# Autodesk Inventor assembly: robot
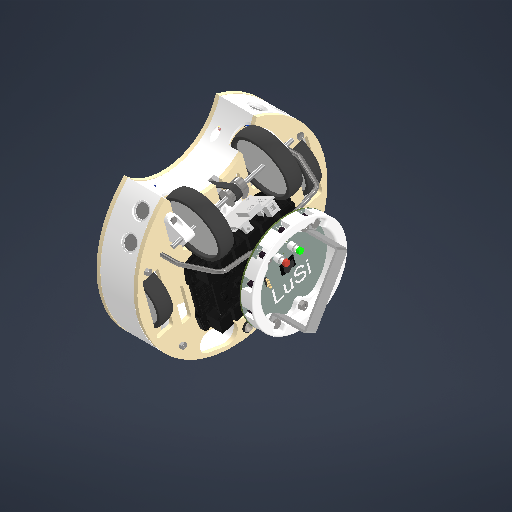
[picture p0: Inventor's stored thumbnail of the model, 512x512]
Saved by Autodesk Inventor 2026.1 (Build 301233000, 233)
## iProperties
Created: 2026-04-20
Part Number: robot
Document SubType Name: Assembly
Designer: Familie
Author: Familie
## Documents named in this file (42)
- C:\Users\Familie\Documents\Luka\Robocup Soccer\Wien\final\robot.iam
- C:\Users\Familie\Documents\Luka\Robocup Soccer\Inventor nach Nürnberg\ball caster.ipt
- C:\Users\Familie\Documents\Luka\Robocup Soccer\Inventor nach Nürnberg\Auriga Steuerboard.ipt
- C:\Users\Familie\Documents\Luka\Robocup Soccer\Inventor nach Nürnberg\Antriebs Rad.ipt
- C:\Users\Familie\Documents\Luka\Robocup Soccer\Inventor nach Nürnberg\Fahrmotor.ipt
- C:\Users\Familie\Documents\Luka\Robocup Soccer\Inventor nach Nürnberg\Mittlere Platte.ipt
- C:\Users\Familie\Documents\Luka\Robocup Soccer\Inventor nach Nürnberg\Grundplatte.ipt
- C:\Users\Familie\Documents\Luka\Robocup Soccer\Inventor nach Nürnberg\Griffroboter.ipt
- C:\Users\Familie\Documents\Luka\Robocup Soccer\Inventor nach Nürnberg\Ultraschalsensor.ipt
- C:\Users\Familie\Documents\Luka\Robocup Soccer\Inventor nach Nürnberg\Umrandung.ipt
- C:\Users\Familie\Documents\Luka\Robocup Soccer\Inventor nach Nürnberg\Halter Ball Caster.ipt
- C:\Users\Familie\Documents\Luka\Robocup Soccer\Inventor nach Nürnberg\IR-Platte.iam
- C:\Users\Familie\Documents\Luka\Robocup Soccer\Inventor nach Nürnberg\Motor Halter.ipt
- C:\Users\Familie\Documents\Inventor\Content Center Files\R2026\de-DE\AS 1110\AS 1110 - M3 x 8.ipt
- C:\Users\Familie\Documents\Inventor\Content Center Files\R2026\de-DE\ANSI B18.2.4.2M\ANSI B18.2.4.2M - M3x0,5 - 5,5.ipt
- C:\Users\Familie\Documents\Inventor\Content Center Files\R2026\de-DE\AS 1110\AS 1110 - M3 x 10.ipt
- C:\Users\Familie\Documents\Inventor\Content Center Files\R2026\de-DE\AS 1110\AS 1110 - M4 x 12.ipt
- C:\Users\Familie\Documents\Inventor\Content Center Files\R2026\de-DE\ANSI B18.2.4.2M\ANSI B18.2.4.2M - M4x0,7 - 7.ipt
- C:\Users\Familie\Documents\Inventor\Content Center Files\R2026\de-DE\AS 1427(03)\AS 1427 - M3 x 6(1).ipt
- C:\Users\Familie\Documents\Luka\KiCad\IR-Platte\Roboter neu\Roboter neu\blue led.ipt
- C:\Users\Familie\Documents\Luka\Robocup Soccer\Inventor nach Nürnberg\LDR\LDR\LDR.ipt
- C:\Users\Familie\Documents\Luka\Robocup Soccer\Inventor nach Nürnberg\Dribbler Motor Halter Oberteil.ipt
- C:\Users\Familie\Documents\Luka\Robocup Soccer\Inventor nach Nürnberg\Dribbler Motor Halter Unterteil.ipt
- C:\Users\Familie\Documents\Luka\Robocup Soccer\Inventor nach Nürnberg\Dribbler Motor.ipt
- C:\Users\Familie\Documents\Luka\Robocup Soccer\Inventor nach Nürnberg\Zahnriemen Rad.ipt
- C:\Users\Familie\Documents\Luka\Robocup Soccer\Inventor\Zahnriemen.ipt
- C:\Users\Familie\Documents\Luka\Robocup Soccer\Inventor nach Nürnberg\Stange Dribbler.ipt
- C:\Users\Familie\Documents\Luka\Robocup Soccer\Inventor nach Nürnberg\Stange Hinten.ipt
- C:\Users\Familie\Documents\Luka\Robocup Soccer\Inventor nach Nürnberg\Stange Vorne.ipt
- C:\Users\Familie\Documents\Luka\Robocup Soccer\Inventor nach Nürnberg\Halter Rolle.ipt
- C:\Users\Familie\Documents\Inventor\Content Center Files\R2026\de-DE\AS 1427(03)\AS 1427 - M3 x 5(1).ipt
- C:\Users\Familie\Documents\Luka\Robocup Soccer\Inventor nach Nürnberg\IR-Blocker.ipt
- C:\Users\Familie\Documents\Inventor\Content Center Files\R2026\de-DE\AS 1110\AS 1110 - M3 x 6.ipt
- C:\Users\Familie\Documents\Luka\Robocup Soccer\Inventor nach Nürnberg\Buchse\Buchse\Buchse.ipt
- C:\Users\Familie\Documents\Luka\Robocup Soccer\Inventor nach Nürnberg\Taster grün.ipt
- C:\Users\Familie\Documents\Luka\Robocup Soccer\Inventor nach Nürnberg\Taster rot.ipt
- C:\Users\Familie\Documents\Luka\Robocup Soccer\Inventor nach Nürnberg\Kippschalter\Kippschalter\Kippschalter.ipt
- C:\Users\Familie\Documents\Inventor\Content Center Files\R2026\de-DE\AS 1110\AS 1110 - M3 x 12.ipt
- C:\Users\Familie\Documents\Inventor\Content Center Files\R2026\de-DE\ANSI B18.2.4.2M\ANSI B18.2.4.2M - M3,5x0,6 - 6.ipt
- C:\Users\Familie\Documents\Luka\Robocup Soccer\Inventor nach Nürnberg\Halter Pixy.ipt
- C:\Users\Familie\Documents\Luka\Robocup Soccer\Inventor nach Nürnberg\Pixy2.ipt
- C:\Users\Familie\Documents\Luka\Robocup Soccer\Inventor nach Nürnberg\Obere Platte.ipt
## Components (107 placed, 41 different names)
1. ball caster:1 — Einfügen:22, Tangential:1, Einfügen:23, Einfügen:24
2. Auriga Steuerboard:1 — Einfügen:69, Winkel:11
3. Antriebs Rad:1 — Einfügen:52
4. Antriebs Rad:2 — Einfügen:51
5. Fahrmotor:1 — Einfügen:45, Einfügen:46, Einfügen:51
6. Fahrmotor:2 — Einfügen:43, Einfügen:44, Einfügen:52
7. Mittlere Platte:1 — Einfügen:62, Einfügen:63, Einfügen:64, Einfügen:65, Einfügen:66, Einfügen:67, Einfügen:68, Einfügen:69, Einfügen:70, Einfügen:72, Winkel:11, Einfügen:74, Einfügen:75, Einfügen:80, Einfügen:81, Einfügen:82, Einfügen:83, Einfügen:89, Einfügen:91, Winkel:12, Einfügen:93, Einfügen:96, Einfügen:101, Einfügen:102, Einfügen:103, Einfügen:104, Einfügen:113, Einfügen:115, Einfügen:117, Einfügen:119, Einfügen:120, Einfügen:121
8. Grundplatte:1 — Passend:1, Passend:2, Passend:3, Passend:4, Passend:5, Passend:6, Passend:7, Passend:8, Passend:9, Passend:10, Passend:11, Passend:12, Einfügen:20, Einfügen:21, Einfügen:25, Einfügen:26, Einfügen:31, Einfügen:32, Einfügen:33, Einfügen:34, Einfügen:35, Einfügen:36, Einfügen:37, Einfügen:38
9. Griffroboter:1 — Einfügen:107, Tangential:8, Einfügen:108, Einfügen:109
10. Umrandung:1 — Passend:1, Passend:12, Passend:13, Passend:14, Winkel:1, Winkel:2, Winkel:3, Winkel:4, Winkel:5, Einfügen:53, Passend:15, Einfügen:54, Passend:16, Einfügen:55, Einfügen:56, Einfügen:57, Einfügen:58, Einfügen:59, Einfügen:60, Einfügen:61, Winkel:6, Winkel:7, Winkel:8, Winkel:9, Winkel:10, Einfügen:62, Einfügen:63
11. Halter Ball Caster:1 — Einfügen:20, Einfügen:21, Einfügen:22, Tangential:1
12. IR-Platte:1 [sub-assembly] — Einfügen:91, Winkel:12, Tangential:5, Tangential:6, Passend:18, Tangential:7, Einfügen:105, Einfügen:106, Passend:20, Passend:21, Passend:22, Einfügen:122
13. Motor Halter:1 — Einfügen:33, Einfügen:34, Einfügen:43, Einfügen:44, Einfügen:49, Einfügen:50
14. Motor Halter:2 — Einfügen:31, Einfügen:32, Einfügen:45, Einfügen:46, Einfügen:47, Einfügen:48
15. AS 1110 - Metrisch M3 x 8:1 — Einfügen:60, Winkel:6
16. AS 1110 - Metrisch M3 x 8:2 — Einfügen:59, Winkel:10
17. AS 1110 - Metrisch M3 x 8:3 — Einfügen:57, Winkel:9
18. AS 1110 - Metrisch M3 x 8:4 — Einfügen:58, Winkel:8
19. AS 1110 - Metrisch M3 x 8:5 — Passend:4, Passend:8, Passend:14, Einfügen:3
20. AS 1110 - Metrisch M3 x 8:6 — Passend:3, Passend:9, Einfügen:18
21. AS 1110 - Metrisch M3 x 8:7 — Passend:2, Passend:10, Passend:13, Einfügen:17
22. AS 1110 - Metrisch M3 x 8:8 — Einfügen:61, Winkel:7
23. AS 1110 - Metrisch M3 x 8:9 — Passend:6, Passend:7, Einfügen:2
24. AS 1110 - Metrisch M3 x 8:10 — Passend:5, Passend:11, Einfügen:19
25. ANSI B18.2.4.2M M3x0,5:1 — Einfügen:68
26. ANSI B18.2.4.2M M3x0,5:2 — Einfügen:66
27. ANSI B18.2.4.2M M3x0,5:3 — Einfügen:67
28. ANSI B18.2.4.2M M3x0,5:4 — Einfügen:65
29. ANSI B18.2.4.2M M3x0,5:5 — Einfügen:64
30. ANSI B18.2.4.2M M3x0,5:6 — Einfügen:19, Winkel:1
31. ANSI B18.2.4.2M M3x0,5:7 — Einfügen:2, Winkel:5
32. ANSI B18.2.4.2M M3x0,5:8 — Einfügen:17, Winkel:2
33. ANSI B18.2.4.2M M3x0,5:9 — Einfügen:3, Winkel:4
34. ANSI B18.2.4.2M M3x0,5:10 — Einfügen:18, Winkel:3
35. ANSI B18.2.4.2M M3x0,5:11 — Einfügen:28
36. ANSI B18.2.4.2M M3x0,5:12 — Einfügen:30
37. ANSI B18.2.4.2M M3x0,5:13 — Einfügen:29
38. ANSI B18.2.4.2M M3x0,5:14 — Einfügen:27
39. AS 1110 - Metrisch M3 x 10:1 — Einfügen:25, Einfügen:27
40. AS 1110 - Metrisch M3 x 10:2 — Einfügen:26, Einfügen:28
41. AS 1110 - Metrisch M3 x 8:11 — Einfügen:24, Einfügen:29
42. AS 1110 - Metrisch M3 x 8:12 — Einfügen:23, Einfügen:30
43. AS 1110 - Metrisch M4 x 12:1 — Einfügen:35, Einfügen:39
44. AS 1110 - Metrisch M4 x 12:2 — Einfügen:36, Einfügen:40
45. AS 1110 - Metrisch M4 x 12:3 — Einfügen:37, Einfügen:41
46. AS 1110 - Metrisch M4 x 12:4 — Einfügen:38, Einfügen:42
47. ANSI B18.2.4.2M M4x0,7:1 — Einfügen:39
48. ANSI B18.2.4.2M M4x0,7:2 — Einfügen:40
49. ANSI B18.2.4.2M M4x0,7:3 — Einfügen:41
50. ANSI B18.2.4.2M M4x0,7:4 — Einfügen:42
51. AS 1427 - Metrisch M3 x 6:1 — Einfügen:48
52. AS 1427 - Metrisch M3 x 6:2 — Einfügen:47
53. AS 1427 - Metrisch M3 x 6:3 — Einfügen:49
54. AS 1427 - Metrisch M3 x 6:4 — Einfügen:50
55. Ultraschalsensor:3 — Einfügen:54, Passend:16
56. Ultraschalsensor:4 — Einfügen:53, Passend:15
57. blue led:1 — Einfügen:55
58. LDR:1 — Einfügen:56
59. AS 1110 - Metrisch M3 x 10:3 — Einfügen:70, Einfügen:71
60. AS 1110 - Metrisch M3 x 10:4 — Einfügen:72, Einfügen:73
61. ANSI B18.2.4.2M M3x0,5:15 — Einfügen:71
62. ANSI B18.2.4.2M M3x0,5:16 — Einfügen:73
63. Dribbler Motor Halter Oberteil:1 — Einfügen:74, Einfügen:75, Passend:17, Fluchtend:1, Fluchtend:2
64. Dribbler Motor Halter Unterteil:1 — Passend:17, Fluchtend:1, Fluchtend:2, Einfügen:76, Tangential:2, Einfügen:78, Einfügen:79
65. Dribbler Motor:1 — Einfügen:76, Tangential:2, Einfügen:77
66. Zahnriemen Rad:1 — Einfügen:87, Einfügen:88
67. Zahnriemen Rad:2 — Einfügen:77, Tangential:3
68. Zahnriemen:1 — Einfügen:88, Tangential:3
69. Stange Dribbler:1 — Einfügen:84, Einfügen:85, Einfügen:86, Einfügen:87
70. Stange Hinten:1 — Einfügen:96, Tangential:7, Einfügen:97, Einfügen:98
71. Stange Vorne:1 — Einfügen:89, Tangential:5, Passend:19, Einfügen:95, Einfügen:99
72. Halter Rolle:1 — Einfügen:80, Einfügen:81, Einfügen:84, Einfügen:112, Einfügen:114
73. Halter Rolle:2 — Einfügen:82, Einfügen:83, Einfügen:116, Einfügen:118
74. Antriebs Rad:3 — Einfügen:85
75. Antriebs Rad:4 — Einfügen:86
76. AS 1427 - Metrisch M3 x 5:1 — Einfügen:78
77. AS 1427 - Metrisch M3 x 5:2 — Einfügen:79
78. Stange Vorne:2 — Einfügen:93, Tangential:6, Einfügen:94, Einfügen:100
79. ANSI B18.2.4.2M M4x0,7:5 — Einfügen:94
80. ANSI B18.2.4.2M M4x0,7:6 — Einfügen:95
81. ANSI B18.2.4.2M M4x0,7:7 — Einfügen:99
82. ANSI B18.2.4.2M M4x0,7:8 — Einfügen:98
83. ANSI B18.2.4.2M M4x0,7:9 — Einfügen:97
84. ANSI B18.2.4.2M M4x0,7:10 — Einfügen:100
85. IR-Blocker:1 — Passend:18, Passend:19, Einfügen:107, Tangential:8
86. AS 1110 - Metrisch M3 x 6:1 — Einfügen:102
87. AS 1110 - Metrisch M3 x 6:2 — Einfügen:101
88. Buchse:1 — Einfügen:104
89. Buchse:2 — Einfügen:103
90. Taster grün:1 — Einfügen:105
91. Taster rot:1 — Einfügen:106
92. Kippschalter:1 — Passend:20, Passend:21, Passend:22, Winkel:13
93. ANSI B18.2.4.2M M4x0,7:11 — Einfügen:110
94. ANSI B18.2.4.2M M4x0,7:12 — Einfügen:111
95. AS 1110 - Metrisch M4 x 12:5 — Einfügen:108, Einfügen:110
96. AS 1110 - Metrisch M4 x 12:6 — Einfügen:109, Einfügen:111
97. AS 1110 - Metrisch M3 x 12:1 — Einfügen:112
98. AS 1110 - Metrisch M3 x 12:2 — Einfügen:114
99. AS 1110 - Metrisch M3 x 12:3 — Einfügen:116
100. AS 1110 - Metrisch M3 x 12:4 — Einfügen:118
101. ANSI B18.2.4.2M M3,5x0,6:1 — Einfügen:113
102. ANSI B18.2.4.2M M3,5x0,6:2 — Einfügen:117
103. ANSI B18.2.4.2M M3,5x0,6:3 — Einfügen:115
104. ANSI B18.2.4.2M M3,5x0,6:4 — Einfügen:119
105. Halter Pixy:1 — Einfügen:120, Einfügen:121, Passend:23, Passend:24
106. Pixy2:1 — Passend:23, Passend:24
107. Obere Platte:1 — Einfügen:122, Winkel:13
## Relationships (152: Insert 106, Mate 24, Angle 13, Tangent 7, Flush 2)
- Passend:1 [Mate]: Grundplatte:1 ↔ Umrandung:1
- Passend:2 [Mate]: Grundplatte:1 ↔ AS 1110 - Metrisch M3 x 8:7
- Passend:3 [Mate]: Grundplatte:1 ↔ AS 1110 - Metrisch M3 x 8:6
- Passend:4 [Mate]: Grundplatte:1 ↔ AS 1110 - Metrisch M3 x 8:5
- Passend:5 [Mate]: Grundplatte:1 ↔ AS 1110 - Metrisch M3 x 8:10
- Passend:6 [Mate]: Grundplatte:1 ↔ AS 1110 - Metrisch M3 x 8:9
- Passend:7 [Mate]: Grundplatte:1 ↔ AS 1110 - Metrisch M3 x 8:9
- Passend:8 [Mate]: Grundplatte:1 ↔ AS 1110 - Metrisch M3 x 8:5
- Passend:9 [Mate]: Grundplatte:1 ↔ AS 1110 - Metrisch M3 x 8:6
- Passend:10 [Mate]: Grundplatte:1 ↔ AS 1110 - Metrisch M3 x 8:7
- Passend:11 [Mate]: Grundplatte:1 ↔ AS 1110 - Metrisch M3 x 8:10
- Passend:12 [Mate]: Grundplatte:1 ↔ Umrandung:1
- Passend:13 [Mate]: Umrandung:1 ↔ AS 1110 - Metrisch M3 x 8:7
- Passend:14 [Mate]: Umrandung:1 ↔ AS 1110 - Metrisch M3 x 8:5
- Einfügen:2 [Insert]: AS 1110 - Metrisch M3 x 8:9 ↔ ANSI B18.2.4.2M M3x0,5:7
- Einfügen:17 [Insert]: AS 1110 - Metrisch M3 x 8:7 ↔ ANSI B18.2.4.2M M3x0,5:8
- Einfügen:3 [Insert]: AS 1110 - Metrisch M3 x 8:5 ↔ ANSI B18.2.4.2M M3x0,5:9
- Einfügen:18 [Insert]: AS 1110 - Metrisch M3 x 8:6 ↔ ANSI B18.2.4.2M M3x0,5:10
- Einfügen:19 [Insert]: AS 1110 - Metrisch M3 x 8:10 ↔ ANSI B18.2.4.2M M3x0,5:6
- Winkel:1 [Angle] (0 deg): Umrandung:1 ↔ ANSI B18.2.4.2M M3x0,5:6
- Winkel:2 [Angle] (0 deg): Umrandung:1 ↔ ANSI B18.2.4.2M M3x0,5:8
- Winkel:3 [Angle] (0 deg): Umrandung:1 ↔ ANSI B18.2.4.2M M3x0,5:10
- Winkel:4 [Angle] (0 deg): Umrandung:1 ↔ ANSI B18.2.4.2M M3x0,5:9
- Winkel:5 [Angle] (0 deg): Umrandung:1 ↔ ANSI B18.2.4.2M M3x0,5:7
- Einfügen:20 [Insert]: Grundplatte:1 ↔ Halter Ball Caster:1
- Einfügen:21 [Insert]: Grundplatte:1 ↔ Halter Ball Caster:1
- Einfügen:22 [Insert]: ball caster:1 ↔ Halter Ball Caster:1
- Tangential:1 (-3 mm): ball caster:1 ↔ Halter Ball Caster:1
- Einfügen:23 [Insert]: ball caster:1 ↔ AS 1110 - Metrisch M3 x 8:12
- Einfügen:24 [Insert]: ball caster:1 ↔ AS 1110 - Metrisch M3 x 8:11
- Einfügen:25 [Insert]: Grundplatte:1 ↔ AS 1110 - Metrisch M3 x 10:1
- Einfügen:26 [Insert]: Grundplatte:1 ↔ AS 1110 - Metrisch M3 x 10:2
- Einfügen:27 [Insert]: ANSI B18.2.4.2M M3x0,5:14 ↔ AS 1110 - Metrisch M3 x 10:1
- Einfügen:28 [Insert]: ANSI B18.2.4.2M M3x0,5:11 ↔ AS 1110 - Metrisch M3 x 10:2
- Einfügen:29 [Insert]: ANSI B18.2.4.2M M3x0,5:13 ↔ AS 1110 - Metrisch M3 x 8:11
- Einfügen:30 [Insert]: ANSI B18.2.4.2M M3x0,5:12 ↔ AS 1110 - Metrisch M3 x 8:12
- Einfügen:31 [Insert]: Grundplatte:1 ↔ Motor Halter:2
- Einfügen:32 [Insert]: Grundplatte:1 ↔ Motor Halter:2
- Einfügen:33 [Insert]: Grundplatte:1 ↔ Motor Halter:1
- Einfügen:34 [Insert]: Grundplatte:1 ↔ Motor Halter:1
- Einfügen:35 [Insert]: Grundplatte:1 ↔ AS 1110 - Metrisch M4 x 12:1
- Einfügen:36 [Insert]: Grundplatte:1 ↔ AS 1110 - Metrisch M4 x 12:2
- Einfügen:37 [Insert]: Grundplatte:1 ↔ AS 1110 - Metrisch M4 x 12:3
- Einfügen:38 [Insert]: Grundplatte:1 ↔ AS 1110 - Metrisch M4 x 12:4
- Einfügen:39 [Insert]: AS 1110 - Metrisch M4 x 12:1 ↔ ANSI B18.2.4.2M M4x0,7:1
- Einfügen:40 [Insert]: AS 1110 - Metrisch M4 x 12:2 ↔ ANSI B18.2.4.2M M4x0,7:2
- Einfügen:41 [Insert]: AS 1110 - Metrisch M4 x 12:3 ↔ ANSI B18.2.4.2M M4x0,7:3
- Einfügen:42 [Insert]: AS 1110 - Metrisch M4 x 12:4 ↔ ANSI B18.2.4.2M M4x0,7:4
- Einfügen:43 [Insert]: Fahrmotor:2 ↔ Motor Halter:1
- Einfügen:44 [Insert]: Fahrmotor:2 ↔ Motor Halter:1
- Einfügen:45 [Insert]: Fahrmotor:1 ↔ Motor Halter:2
- Einfügen:46 [Insert]: Fahrmotor:1 ↔ Motor Halter:2
- Einfügen:47 [Insert] (-1 mm): Motor Halter:2 ↔ AS 1427 - Metrisch M3 x 6:2
- Einfügen:48 [Insert] (-1 mm): Motor Halter:2 ↔ AS 1427 - Metrisch M3 x 6:1
- Einfügen:49 [Insert] (-1 mm): Motor Halter:1 ↔ AS 1427 - Metrisch M3 x 6:3
- Einfügen:50 [Insert] (-1 mm): Motor Halter:1 ↔ AS 1427 - Metrisch M3 x 6:4
- Einfügen:51 [Insert] (-1 mm): Antriebs Rad:2 ↔ Fahrmotor:1
- Einfügen:52 [Insert] (-1 mm): Antriebs Rad:1 ↔ Fahrmotor:2
- Einfügen:53 [Insert] (-1 mm): Umrandung:1 ↔ Ultraschalsensor:4
- Passend:15 [Mate]: Umrandung:1 ↔ Ultraschalsensor:4
- Einfügen:54 [Insert] (-1 mm): Umrandung:1 ↔ Ultraschalsensor:3
- Passend:16 [Mate]: Umrandung:1 ↔ Ultraschalsensor:3
- Einfügen:55 [Insert] (6 mm): Umrandung:1 ↔ blue led:1
- Einfügen:56 [Insert] (2 mm): Umrandung:1 ↔ LDR:1
- Einfügen:57 [Insert]: Umrandung:1 ↔ AS 1110 - Metrisch M3 x 8:3
- Einfügen:58 [Insert]: Umrandung:1 ↔ AS 1110 - Metrisch M3 x 8:4
- Einfügen:59 [Insert]: Umrandung:1 ↔ AS 1110 - Metrisch M3 x 8:2
- Einfügen:60 [Insert]: Umrandung:1 ↔ AS 1110 - Metrisch M3 x 8:1
- Einfügen:61 [Insert]: Umrandung:1 ↔ AS 1110 - Metrisch M3 x 8:8
- Winkel:6 [Angle] (0 deg): Umrandung:1 ↔ AS 1110 - Metrisch M3 x 8:1
- Winkel:7 [Angle] (0 deg): Umrandung:1 ↔ AS 1110 - Metrisch M3 x 8:8
- Winkel:8 [Angle] (0 deg): Umrandung:1 ↔ AS 1110 - Metrisch M3 x 8:4
- Winkel:9 [Angle] (0 deg): Umrandung:1 ↔ AS 1110 - Metrisch M3 x 8:3
- Winkel:10 [Angle] (0 deg): Umrandung:1 ↔ AS 1110 - Metrisch M3 x 8:2
- Einfügen:62 [Insert]: Mittlere Platte:1 ↔ Umrandung:1
- Einfügen:63 [Insert]: Mittlere Platte:1 ↔ Umrandung:1
- Einfügen:64 [Insert]: Mittlere Platte:1 ↔ ANSI B18.2.4.2M M3x0,5:5
- Einfügen:65 [Insert]: Mittlere Platte:1 ↔ ANSI B18.2.4.2M M3x0,5:4
- Einfügen:66 [Insert]: Mittlere Platte:1 ↔ ANSI B18.2.4.2M M3x0,5:2
- Einfügen:67 [Insert]: Mittlere Platte:1 ↔ ANSI B18.2.4.2M M3x0,5:3
- Einfügen:68 [Insert]: Mittlere Platte:1 ↔ ANSI B18.2.4.2M M3x0,5:1
- Einfügen:69 [Insert] (2.7 mm): Auriga Steuerboard:1 ↔ Mittlere Platte:1
- Einfügen:70 [Insert]: Mittlere Platte:1 ↔ AS 1110 - Metrisch M3 x 10:3
- Einfügen:71 [Insert] (0.3 mm): AS 1110 - Metrisch M3 x 10:3 ↔ ANSI B18.2.4.2M M3x0,5:15
- Einfügen:72 [Insert]: Mittlere Platte:1 ↔ AS 1110 - Metrisch M3 x 10:4
- Einfügen:73 [Insert] (-0.3 mm): AS 1110 - Metrisch M3 x 10:4 ↔ ANSI B18.2.4.2M M3x0,5:16
- Winkel:11 [Angle] (0 deg): Auriga Steuerboard:1 ↔ Mittlere Platte:1
- Einfügen:74 [Insert]: Mittlere Platte:1 ↔ Dribbler Motor Halter Oberteil:1
- Einfügen:75 [Insert]: Mittlere Platte:1 ↔ Dribbler Motor Halter Oberteil:1
- Passend:17 [Mate]: Dribbler Motor Halter Oberteil:1 ↔ Dribbler Motor Halter Unterteil:1
- Fluchtend:1 [Flush]: Dribbler Motor Halter Oberteil:1 ↔ Dribbler Motor Halter Unterteil:1
- Fluchtend:2 [Flush]: Dribbler Motor Halter Oberteil:1 ↔ Dribbler Motor Halter Unterteil:1
- Einfügen:76 [Insert]: Dribbler Motor Halter Unterteil:1 ↔ Dribbler Motor:1
- Tangential:2: Dribbler Motor Halter Unterteil:1 ↔ Dribbler Motor:1
- Einfügen:77 [Insert] (-6 mm): Dribbler Motor:1 ↔ Zahnriemen Rad:2
- Einfügen:78 [Insert] (0.2 mm): Dribbler Motor Halter Unterteil:1 ↔ AS 1427 - Metrisch M3 x 5:1
- Einfügen:79 [Insert] (-0.2 mm): Dribbler Motor Halter Unterteil:1 ↔ AS 1427 - Metrisch M3 x 5:2
- Einfügen:80 [Insert]: Mittlere Platte:1 ↔ Halter Rolle:1
- Einfügen:81 [Insert]: Mittlere Platte:1 ↔ Halter Rolle:1
- Einfügen:82 [Insert]: Mittlere Platte:1 ↔ Halter Rolle:2
- Einfügen:83 [Insert]: Mittlere Platte:1 ↔ Halter Rolle:2
- Einfügen:84 [Insert] (-9.25 mm): Stange Dribbler:1 ↔ Halter Rolle:1
- Einfügen:85 [Insert] (-32 mm): Stange Dribbler:1 ↔ Antriebs Rad:3
- Einfügen:86 [Insert] (-32 mm): Stange Dribbler:1 ↔ Antriebs Rad:4
- Einfügen:87 [Insert] (-72 mm): Zahnriemen Rad:1 ↔ Stange Dribbler:1
- Einfügen:88 [Insert] (1.3 mm): Zahnriemen Rad:1 ↔ Zahnriemen:1
- Tangential:3 (-11.1 mm): Zahnriemen Rad:2 ↔ Zahnriemen:1
- Einfügen:89 [Insert] (3 mm): Mittlere Platte:1 ↔ Stange Vorne:1
- Einfügen:91 [Insert] (57.5 mm): Mittlere Platte:1 ↔ IR-Platte:1
- Winkel:12 [Angle] (0 deg): Mittlere Platte:1 ↔ IR-Platte:1
- Einfügen:93 [Insert] (3 mm): Mittlere Platte:1 ↔ Stange Vorne:2
- Tangential:5 (-3.9 mm): IR-Platte:1 ↔ Stange Vorne:1
- Tangential:6 (-3.89 mm): IR-Platte:1 ↔ Stange Vorne:2
- Passend:18 [Mate]: IR-Platte:1 ↔ IR-Blocker:1
- Passend:19 [Mate]: Stange Vorne:1 ↔ IR-Blocker:1
- Einfügen:94 [Insert]: Stange Vorne:2 ↔ ANSI B18.2.4.2M M4x0,7:5
- Einfügen:95 [Insert]: Stange Vorne:1 ↔ ANSI B18.2.4.2M M4x0,7:6
- Einfügen:96 [Insert] (-3 mm): Mittlere Platte:1 ↔ Stange Hinten:1
- Tangential:7 (-3.9 mm): IR-Platte:1 ↔ Stange Hinten:1
- Einfügen:97 [Insert] (-0.9 mm): Stange Hinten:1 ↔ ANSI B18.2.4.2M M4x0,7:9
- Einfügen:98 [Insert]: Stange Hinten:1 ↔ ANSI B18.2.4.2M M4x0,7:8
- Einfügen:99 [Insert]: Stange Vorne:1 ↔ ANSI B18.2.4.2M M4x0,7:7
- Einfügen:100 [Insert]: Stange Vorne:2 ↔ ANSI B18.2.4.2M M4x0,7:10
- Einfügen:101 [Insert]: Mittlere Platte:1 ↔ AS 1110 - Metrisch M3 x 6:2
- Einfügen:102 [Insert]: Mittlere Platte:1 ↔ AS 1110 - Metrisch M3 x 6:1
- Einfügen:103 [Insert] (-2 mm): Mittlere Platte:1 ↔ Buchse:2
- Einfügen:104 [Insert] (-2 mm): Mittlere Platte:1 ↔ Buchse:1
- Einfügen:105 [Insert]: IR-Platte:1 ↔ Taster grün:1
- Einfügen:106 [Insert]: IR-Platte:1 ↔ Taster rot:1
- Passend:20 [Mate] (1 mm): IR-Platte:1 ↔ Kippschalter:1
- Passend:21 [Mate] (1.5 mm): IR-Platte:1 ↔ Kippschalter:1
- Passend:22 [Mate] (-0.2 mm): IR-Platte:1 ↔ Kippschalter:1
- Einfügen:107 [Insert]: Griffroboter:1 ↔ IR-Blocker:1
- Tangential:8 (-3.9 mm): Griffroboter:1 ↔ IR-Blocker:1
- Einfügen:108 [Insert]: Griffroboter:1 ↔ AS 1110 - Metrisch M4 x 12:5
- Einfügen:109 [Insert]: Griffroboter:1 ↔ AS 1110 - Metrisch M4 x 12:6
- Einfügen:110 [Insert] (-0.5 mm): ANSI B18.2.4.2M M4x0,7:11 ↔ AS 1110 - Metrisch M4 x 12:5
- Einfügen:111 [Insert] (-0.5 mm): ANSI B18.2.4.2M M4x0,7:12 ↔ AS 1110 - Metrisch M4 x 12:6
- Einfügen:112 [Insert]: Halter Rolle:1 ↔ AS 1110 - Metrisch M3 x 12:1
- Einfügen:113 [Insert]: Mittlere Platte:1 ↔ ANSI B18.2.4.2M M3,5x0,6:1
- Einfügen:114 [Insert]: Halter Rolle:1 ↔ AS 1110 - Metrisch M3 x 12:2
- Einfügen:115 [Insert]: Mittlere Platte:1 ↔ ANSI B18.2.4.2M M3,5x0,6:3
- Einfügen:116 [Insert]: Halter Rolle:2 ↔ AS 1110 - Metrisch M3 x 12:3
- Einfügen:117 [Insert]: Mittlere Platte:1 ↔ ANSI B18.2.4.2M M3,5x0,6:2
- Einfügen:118 [Insert]: Halter Rolle:2 ↔ AS 1110 - Metrisch M3 x 12:4
- Einfügen:119 [Insert]: Mittlere Platte:1 ↔ ANSI B18.2.4.2M M3,5x0,6:4
- Einfügen:120 [Insert]: Mittlere Platte:1 ↔ Halter Pixy:1
- Einfügen:121 [Insert]: Mittlere Platte:1 ↔ Halter Pixy:1
- Passend:23 [Mate]: Halter Pixy:1 ↔ Pixy2:1
- Passend:24 [Mate]: Halter Pixy:1 ↔ Pixy2:1
- Einfügen:122 [Insert]: IR-Platte:1 ↔ Obere Platte:1
- Winkel:13 [Angle] (0 deg): Kippschalter:1 ↔ Obere Platte:1
